# Autodesk Inventor assembly: A002
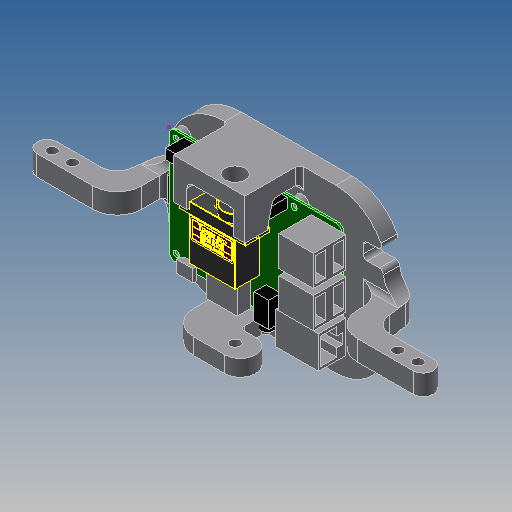
[picture p0: Inventor's stored thumbnail of the model, 512x512]
Saved by Autodesk Inventor 2017 (Build 210142000, 142)
## iProperties
Created: 2018-10-19
Part Number: A002
Document SubType Name: Assembly
Designer: Gilles Mottiez
Description: Plateforme mobile
Author: Gilles Mottiez
## Documents named in this file (6)
- C:\Users\Gilles Mottiez\Documents\HES\I5_6\PGA\inventor\plateforme_rpi_servo.iam
- plateforme_rpi_servo.iam
- C:\Users\Gilles Mottiez\Documents\HES\I5_6\PGA\inventor\plateforme_rpi_servo_new.ipt
- plateforme_rpi_servo_new.ipt
- C:\Users\Gilles Mottiez\Documents\HES\I5_6\PGA\inventor\rpi3b.iam
- C:\Users\Gilles Mottiez\Documents\HES\I5_6\PGA\inventor\MG90s_servo.ipt
## Components (3 placed, 3 different names)
1. plateforme_rpi_servo_new:1 — Logement:1, Logement:2, Placage:1, Placage:2, Angle:1
2. rpi3b:1 [sub-assembly] — Logement:1, Logement:2
3. MG90s_servo:1 — Placage:1, Placage:2, Angle:1
## Relationships (5: Insert 2, Mate 2, Angle 1)
- Logement:1 [Insert]: plateforme_rpi_servo_new:1 ↔ rpi3b:1
- Logement:2 [Insert]: plateforme_rpi_servo_new:1 ↔ rpi3b:1
- Placage:1 [Mate]: plateforme_rpi_servo_new:1 ↔ MG90s_servo:1
- Placage:2 [Mate]: plateforme_rpi_servo_new:1 ↔ MG90s_servo:1
- Angle:1 (0 deg): plateforme_rpi_servo_new:1 ↔ MG90s_servo:1
